# Autodesk Inventor assembly: Shooter-Storage-IntakeAssembly.ver1-1111-2021
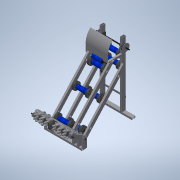
[picture p0: Inventor's stored thumbnail of the model, 180x180]
Saved by Autodesk Inventor 2021 (Build 250183000, 183)
## iProperties
Created: 2020-01-25
Part Number: Shooter-Storage-IntakeAssembly.ver1-1111-2021
Document SubType Name: Assembly
Designer: JMHal
Author: JMHal
## Documents named in this file (6)
- E:\PHRC CADD 2021\PHRC CADD\2020 Infinite Recharge\2021 Infinite Recharge\Chassis\Shooter-Storage-IntakeAssembly.ver1-1111-2021.iam
- E:\PHRC CADD 2021\PHRC CADD\2020 Infinite Recharge\Final Robot Assembly\IntakeAssembly-ver1-1111-2020.iam
- E:\PHRC CADD 2021\PHRC CADD\2020 Infinite Recharge\Shooting\Assemblies\ShooterPrototype-ver2-1111-2019.iam
- E:\PHRC CADD 2021\PHRC CADD\2020 Infinite Recharge\Storage\Assemblies\StorageAssembly.ver4-1111-2020.iam
- E:\PHRC CADD 2021\PHRC CADD\2020 Infinite Recharge\Storage\Assemblies\Roller-ver1-1111-2019.iam
- E:\PHRC CADD 2021\PHRC CADD\2020 Infinite Recharge\Storage\Assemblies\TopRoller-ver1-1111-2019.iam
## Components (12 placed, 5 different names)
1. IntakeAssembly-ver1-1111-2020:1 [sub-assembly] — Flush:2, Mate:3, Mate:8
2. ShooterPrototype-ver2-1111-2019:1 [sub-assembly] — Mate:2, Cylindrical:6, Mate:4, Mate:5, Cylindrical:8, Mate:7
3. StorageAssembly.ver4-1111-2020:1 [sub-assembly] — Mate:2, Flush:2, Mate:3, Cylindrical:4, Cylindrical:5, Mate:5, Mate:6, Cylindrical:9, Cylindrical:10, Cylindrical:11, Mate:8, Cylindrical:12
4. Roller-ver1-1111-2019:1 [sub-assembly] — Cylindrical:11, Flush:4, Flush:5, Flush:8
5. Roller-ver1-1111-2019:2 [sub-assembly] — Flush:5, Flush:6
6. Roller-ver1-1111-2019:4 [sub-assembly] — Cylindrical:4, Flush:6, Flush:7
7. Roller-ver1-1111-2019:5 [sub-assembly] — Cylindrical:5, Flush:8
8. Roller-ver1-1111-2019:6 [sub-assembly] — Cylindrical:6, Mate:4
9. TopRoller-ver1-1111-2019:1 [sub-assembly] — Mate:6, Cylindrical:9, Flush:3
10. Roller-ver1-1111-2019:7 [sub-assembly] — Cylindrical:8, Mate:7, Flush:9
11. Roller-ver1-1111-2019:8 [sub-assembly] — Cylindrical:10, Flush:3, Flush:4, Flush:9
12. TopRoller-ver1-1111-2019:2 [sub-assembly] — Cylindrical:12, Flush:7
## Relationships (23: Flush 8, CylindricalJoint 8, Mate 7)
- Mate:2: ShooterPrototype-ver2-1111-2019:1 ↔ StorageAssembly.ver4-1111-2020:1
- Flush:2: IntakeAssembly-ver1-1111-2020:1 ↔ StorageAssembly.ver4-1111-2020:1
- Mate:3: IntakeAssembly-ver1-1111-2020:1 ↔ StorageAssembly.ver4-1111-2020:1
- Cylindrical:4: StorageAssembly.ver4-1111-2020:1 ↔ Roller-ver1-1111-2019:4
- Cylindrical:5: StorageAssembly.ver4-1111-2020:1 ↔ Roller-ver1-1111-2019:5
- Cylindrical:6: ShooterPrototype-ver2-1111-2019:1 ↔ Roller-ver1-1111-2019:6
- Mate:4 (3.175 mm): ShooterPrototype-ver2-1111-2019:1 ↔ Roller-ver1-1111-2019:6
- Mate:5: ShooterPrototype-ver2-1111-2019:1 ↔ StorageAssembly.ver4-1111-2020:1
- Mate:6 (28.575 mm): StorageAssembly.ver4-1111-2020:1 ↔ TopRoller-ver1-1111-2019:1
- Cylindrical:8: ShooterPrototype-ver2-1111-2019:1 ↔ Roller-ver1-1111-2019:7
- Mate:7 (3.175 mm): ShooterPrototype-ver2-1111-2019:1 ↔ Roller-ver1-1111-2019:7
- Cylindrical:9: StorageAssembly.ver4-1111-2020:1 ↔ TopRoller-ver1-1111-2019:1
- Cylindrical:10: StorageAssembly.ver4-1111-2020:1 ↔ Roller-ver1-1111-2019:8
- Cylindrical:11: StorageAssembly.ver4-1111-2020:1 ↔ Roller-ver1-1111-2019:1
- Mate:8 (64.7065 mm): IntakeAssembly-ver1-1111-2020:1 ↔ StorageAssembly.ver4-1111-2020:1
- Cylindrical:12: StorageAssembly.ver4-1111-2020:1 ↔ TopRoller-ver1-1111-2019:2
- Flush:3: TopRoller-ver1-1111-2019:1 ↔ Roller-ver1-1111-2019:8
- Flush:4: Roller-ver1-1111-2019:1 ↔ Roller-ver1-1111-2019:8
- Flush:5: Roller-ver1-1111-2019:1 ↔ Roller-ver1-1111-2019:2
- Flush:6: Roller-ver1-1111-2019:2 ↔ Roller-ver1-1111-2019:4
- Flush:7: Roller-ver1-1111-2019:4 ↔ TopRoller-ver1-1111-2019:2
- Flush:8: Roller-ver1-1111-2019:1 ↔ Roller-ver1-1111-2019:5
- Flush:9: Roller-ver1-1111-2019:7 ↔ Roller-ver1-1111-2019:8
